# Autodesk Inventor assembly: solarCar
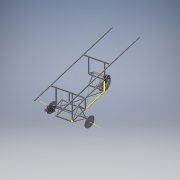
[picture p0: Inventor's stored thumbnail of the model, 180x180]
Saved by Autodesk Inventor 2018 (Build 220112000, 112)
## iProperties
Created: 2018-03-20
Part Number: solarCar
Document SubType Name: Assembly
Designer: rochee19
Author: rochee19
## Documents named in this file (7)
- C:\Users\andrecheke21\Desktop\SolarCarCAD\solarCar.iam
- C:\Users\andrecheke21\Desktop\SolarCarCAD\finalDoneskies.ipt
- C:\Users\andrecheke21\Desktop\SolarCarCAD\lefttURNwHEEL.iam
- C:\Users\andrecheke21\Desktop\SolarCarCAD\rearWheel.ipt
- C:\Users\andrecheke21\Desktop\SolarCarCAD\righttURNwHEEL.iam
- C:\Users\andrecheke21\Desktop\SolarCarCAD\stableBar.ipt
- C:\Users\andrecheke21\Desktop\SolarCarCAD\RearCrumple.ipt
## Components (6 placed, 6 different names)
1. finalDoneskies:1 — Insert:5, Insert:6, Flush:2, Flush:4, Flush:5, Flush:6, Mate:1, Mate:2
2. rearWheel:1
3. lefttURNwHEEL:1 [sub-assembly] — Insert:5, Insert:8
4. righttURNwHEEL:1 [sub-assembly] — Insert:6, Insert:7
5. stableBar:1 — Insert:7, Insert:8
6. RearCrumple:1 — Flush:2, Flush:4, Flush:5, Flush:6, Mate:1, Mate:2
## Relationships (10: Insert 4, Flush 4, Mate 2)
- Insert:5: finalDoneskies:1 ↔ lefttURNwHEEL:1
- Insert:6: finalDoneskies:1 ↔ righttURNwHEEL:1
- Insert:7: righttURNwHEEL:1 ↔ stableBar:1
- Insert:8: lefttURNwHEEL:1 ↔ stableBar:1
- Flush:2: finalDoneskies:1 ↔ RearCrumple:1
- Flush:4: finalDoneskies:1 ↔ RearCrumple:1
- Flush:5: finalDoneskies:1 ↔ RearCrumple:1
- Flush:6: finalDoneskies:1 ↔ RearCrumple:1
- Mate:1: finalDoneskies:1 ↔ RearCrumple:1
- Mate:2: finalDoneskies:1 ↔ RearCrumple:1
